# Autodesk Inventor assembly: Matchboxscope_v0
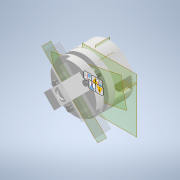
[picture p0: Inventor's stored thumbnail of the model, 180x180]
Saved by Autodesk Inventor 2022 (Build 260153000, 153)
## iProperties
Created: 2022-03-21
Part Number: Matchboxscope_v0
Document SubType Name: Assembly
Designer: Prakash Lab
Author: Prakash Lab
## Documents named in this file (10)
- C:\Users\PrakashLab\Documents\Matchboxscope\INVENTOR\Matchboxscope_v0.iam
- C:\Users\PrakashLab\Documents\Matchboxscope\INVENTOR\Matchboxscope_bottom_v0.ipt
- C:\Users\PrakashLab\Documents\Matchboxscope\INVENTOR\Matchboxscope_middle2_v1.ipt
- C:\Users\PrakashLab\Documents\Matchboxscope\INVENTOR\00_ESP3-CAM.iam
- C:\Users\PrakashLab\Documents\Matchboxscope\INVENTOR\camera for ESP32 v1.iam
- C:\Users\PrakashLab\Documents\Matchboxscope\INVENTOR\00_chip.ipt
- C:\Users\PrakashLab\Documents\Matchboxscope\INVENTOR\Matchboxscope_sample_v0.ipt
- C:\Users\PrakashLab\Documents\Matchboxscope\INVENTOR\Matchboxscope_lenstube_v0.ipt
- C:\Users\PrakashLab\Documents\Matchboxscope\INVENTOR\Matchboxscope_Lightperiscope_V0.ipt
- C:\Users\PrakashLab\Documents\Inventor\Content Center Files\R2022\en-US\DIN 912\DIN 912 - M3 x 0.5 x 20 x 18.75.ipt
## Components (17 placed, 9 different names)
1. Matchboxscope_bottom_v0:1 — Mate:1, Flush:1, Mate:2, Mate:20, Insert:1, Flush:3, Mate:23, Mate:25, Insert:5, Insert:6, Insert:7, Insert:8
2. Matchboxscope_lenstube_v0:1 — Insert:2
3. 00_ESP3-CAM:5 [sub-assembly] — Mate:20, Mate:22, Flush:3
4. camera for ESP32 v1:3 [sub-assembly] — Mate:21, Insert:2
5. Matchboxscope_middle2_v1:1 — Insert:1, Mate:21, Mate:22, Insert:3
6. 00_chip:1 — Mate:23, Mate:24, Mate:25
7. Matchboxscope_sample_v0:1 — Insert:3, Insert:4, Mate:24, Insert:9, Insert:10, Insert:11
8. Matchboxscope_Lightperiscope_V0:1 — Insert:4
9. DIN 912 - replaced by DIN EN ISO 4762 M3 x 20:1 — Insert:7
10. DIN 912 - replaced by DIN EN ISO 4762 M3 x 20:2 — Insert:6
11. DIN 912 - replaced by DIN EN ISO 4762 M3 x 20:3 — Insert:5
12. DIN 912 - replaced by DIN EN ISO 4762 M3 x 20:4 — Insert:8
13. DIN 912 - replaced by DIN EN ISO 4762 M3 x 20:5 — Insert:10
14. DIN 912 - replaced by DIN EN ISO 4762 M3 x 20:6 — Insert:11
15. DIN 912 - replaced by DIN EN ISO 4762 M3 x 20:9 — Insert:9
16. 00_ESP3-CAM:1 [sub-assembly] — Mate:1, Flush:1
17. 00_ESP3-CAM:3 [sub-assembly] — Mate:2
## Component patterns: (2 elements, first: 00_ESP3-CAM:1)
## Relationships (22: Insert 11, Mate 9, Flush 2)
- Mate:1: Matchboxscope_bottom_v0:1 ↔ 00_ESP3-CAM:1
- Flush:1: Matchboxscope_bottom_v0:1 ↔ 00_ESP3-CAM:1
- Mate:2 (1 mm): Matchboxscope_bottom_v0:1 ↔ 00_ESP3-CAM:3
- [Mate]: 00_ESP3-CAM:5 ↔ camera for ESP32 v1:3
- Mate:20: Matchboxscope_bottom_v0:1 ↔ 00_ESP3-CAM:5
- Insert:1: Matchboxscope_bottom_v0:1 ↔ Matchboxscope_middle2_v1:1
- Mate:21: camera for ESP32 v1:3 ↔ Matchboxscope_middle2_v1:1
- Mate:22 (3 mm): 00_ESP3-CAM:5 ↔ Matchboxscope_middle2_v1:1
- Flush:3: Matchboxscope_bottom_v0:1 ↔ 00_ESP3-CAM:5
- Insert:2 (-2 mm): Matchboxscope_lenstube_v0:1 ↔ camera for ESP32 v1:3
- Insert:3 (5 mm): Matchboxscope_middle2_v1:1 ↔ Matchboxscope_sample_v0:1
- Insert:4: Matchboxscope_sample_v0:1 ↔ Matchboxscope_Lightperiscope_V0:1
- Mate:23: Matchboxscope_bottom_v0:1 ↔ 00_chip:1
- Mate:24: 00_chip:1 ↔ Matchboxscope_sample_v0:1
- Mate:25 (-40 mm): Matchboxscope_bottom_v0:1 ↔ 00_chip:1
- Insert:5: Matchboxscope_bottom_v0:1 ↔ DIN 912 - replaced by DIN EN ISO 4762 M3 x 20:3
- Insert:6: Matchboxscope_bottom_v0:1 ↔ DIN 912 - replaced by DIN EN ISO 4762 M3 x 20:2
- Insert:7: Matchboxscope_bottom_v0:1 ↔ DIN 912 - replaced by DIN EN ISO 4762 M3 x 20:1
- Insert:8: Matchboxscope_bottom_v0:1 ↔ DIN 912 - replaced by DIN EN ISO 4762 M3 x 20:4
- Insert:9: Matchboxscope_sample_v0:1 ↔ DIN 912 - replaced by DIN EN ISO 4762 M3 x 20:9
- Insert:10: Matchboxscope_sample_v0:1 ↔ DIN 912 - replaced by DIN EN ISO 4762 M3 x 20:5
- Insert:11: Matchboxscope_sample_v0:1 ↔ DIN 912 - replaced by DIN EN ISO 4762 M3 x 20:6
## Named parameters: d50_d24 = 0 mm
